# Autodesk Inventor assembly: Gearbox Assembly
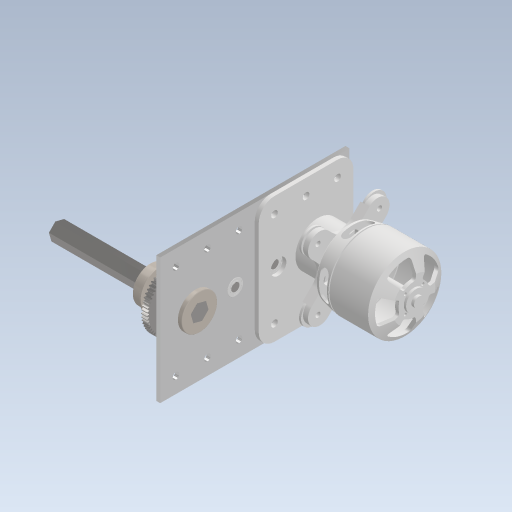
[picture p0: Inventor's stored thumbnail of the model, 512x512]
Saved by Autodesk Inventor 2023 (Build 270158000, 158)
## iProperties
Created: 2023-02-14
Part Number: Gearbox Assembly
Document SubType Name: Assembly
Designer: Dave
Mass: 682.162 g
Surface Area: 1267.39 cm^2
Volume: 183.282 cm^3
Density: 3.72192 g/cm^3
Author: Dave
## Documents named in this file (14)
- C:\Users\Dave\Documents\GitHub\BehrendURCMechanical\CAD\Chassis\GearBox\Final Gears and Assemblies\Gearbox Assembly.iam
- C:\Users\Dave\Documents\GitHub\BehrendURCMechanical\CAD\Chassis\GearBox\Final Gears and Assemblies\CH-1-01-20T_Drive Gear.ipt
- C:\Users\Dave\Documents\GitHub\BehrendURCMechanical\CAD\Chassis\GearBox\Final Gears and Assemblies\CH-1-01-60T_Output.ipt
- C:\Users\Dave\Documents\GitHub\BehrendURCMechanical\CAD\Chassis\GearBox\Final Gears and Assemblies\CH-1-01-20T_Idler.ipt
- C:\Users\Dave\Documents\GitHub\BehrendURCMechanical\CAD\Chassis\GearBox\Final Gears and Assemblies\CH-1-01-60T_Idler.ipt
- C:\Users\Dave\Documents\GitHub\BehrendURCMechanical\CAD\Chassis\GearBox\Housing\CH-1-02-RearGearboxHousingMotorSide.ipt
- C:\Users\Dave\Documents\GitHub\BehrendURCMechanical\CAD\Chassis\GearBox\Drive Motor Shaft Coupler.ipt
- C:\Users\Dave\Documents\GitHub\BehrendURCMechanical\CAD\Chassis\GearBox\Drive Motor.ipt
- C:\Users\Dave\Documents\GitHub\BehrendURCMechanical\CAD\Chassis\GearBox\Ch-1-01-0.5x4.5HexShaft.ipt
- C:\Users\Dave\Documents\GitHub\BehrendURCMechanical\CAD\Chassis\GearBox\CH-1-01-0.25x1.875SmoothShaft.ipt
- C:\Users\Dave\Documents\GitHub\BehrendURCMechanical\CAD\Chassis\GearBox\CH-1-01-0.5HexBearing.ipt
- C:\Users\Dave\Documents\GitHub\BehrendURCMechanical\CAD\Chassis\GearBox\CH-1-01-0.25IDSmoothBoreBearing.ipt
- C:\Users\Dave\Documents\GitHub\BehrendURCMechanical\CAD\Chassis V3\DriveMotorPlate.ipt
- C:\Users\Dave\Documents\GitHub\BehrendURCMechanical\CAD\Chassis V3\DriveMotorMount2.ipt
## Components (21 placed, 13 different names)
1. CH-1-01-20T_Drive Gear:1 — Insert:3
2. CH-1-01-60T_Output:1 — Mate:17, Flush:6
3. CH-1-01-20T_Idler:1 — Mate:21, Flush:5
4. CH-1-01-60T_Idler:1 — Mate:18, Mate:19, Mate:20, Flush:5
5. CH-1-01-20T_Idler:2 — Mate:19, Mate:22, Flush:6
6. CH-1-01-60T_Idler:2 — Mate:10, Mate:11, Mate:23
7. CH-1-02-RearGearboxHousingMotorSide:1 — Angle:1, Flush:1, Flush:2, Insert:6, Insert:7, Insert:10, Mate:26, Angle:2, Flush:8, Flush:9
8. CH-1-02-RearGearboxHousingMotorSide:2 — Flush:1, Flush:2, Insert:8, Insert:9, Insert:11
9. Drive Motor Shaft Coupler:1 — Insert:3, Mate:23, Mate:24, Mate:25, Flush:7, Mate:26
10. Drive Motor:1 — Mate:24, Mate:25, Angle:2, Insert:14, Insert:15
11. Ch-1-01-0.5x4.5HexShaft:1 — Flush:3, Mate:8, Mate:9
12. CH-1-01-0.25x1.875SmoothShaft:1 — Insert:13
13. CH-1-01-0.25x1.875SmoothShaft:2 — Insert:12, Flush:4
14. CH-1-01-0.5HexBearing:1 — Insert:11, Mate:17
15. CH-1-01-0.5HexBearing:2 — Insert:10, Flush:3, Mate:8, Mate:9
16. CH-1-01-0.25IDSmoothBoreBearing:1 — Insert:6, Insert:12, Flush:7
17. CH-1-01-0.25IDSmoothBoreBearing:2 — Insert:7, Insert:13, Mate:11
18. CH-1-01-0.25IDSmoothBoreBearing:3 — Insert:8, Flush:4, Mate:18, Mate:20, Mate:22
19. CH-1-01-0.25IDSmoothBoreBearing:4 — Insert:9, Mate:10, Mate:21
20. DriveMotorPlate:1 — Insert:14, Insert:15, Flush:10
21. DriveMotorMount2:1 — Flush:8, Flush:9, Flush:10
## Relationships (37: Mate 14, Insert 11, Flush 10, Angle 2)
- Insert:3: CH-1-01-20T_Drive Gear:1 ↔ Drive Motor Shaft Coupler:1
- Angle:1 (0 deg): CH-1-02-RearGearboxHousingMotorSide:1
- Flush:1: CH-1-02-RearGearboxHousingMotorSide:1 ↔ CH-1-02-RearGearboxHousingMotorSide:2
- Flush:2: CH-1-02-RearGearboxHousingMotorSide:1 ↔ CH-1-02-RearGearboxHousingMotorSide:2
- Insert:6: CH-1-02-RearGearboxHousingMotorSide:1 ↔ CH-1-01-0.25IDSmoothBoreBearing:1
- Insert:7: CH-1-02-RearGearboxHousingMotorSide:1 ↔ CH-1-01-0.25IDSmoothBoreBearing:2
- Insert:8: CH-1-02-RearGearboxHousingMotorSide:2 ↔ CH-1-01-0.25IDSmoothBoreBearing:3
- Insert:9: CH-1-02-RearGearboxHousingMotorSide:2 ↔ CH-1-01-0.25IDSmoothBoreBearing:4
- Insert:10: CH-1-02-RearGearboxHousingMotorSide:1 ↔ CH-1-01-0.5HexBearing:2
- Insert:11: CH-1-02-RearGearboxHousingMotorSide:2 ↔ CH-1-01-0.5HexBearing:1
- Flush:3: Ch-1-01-0.5x4.5HexShaft:1 ↔ CH-1-01-0.5HexBearing:2
- Mate:8: Ch-1-01-0.5x4.5HexShaft:1 ↔ CH-1-01-0.5HexBearing:2
- Mate:9: Ch-1-01-0.5x4.5HexShaft:1 ↔ CH-1-01-0.5HexBearing:2
- Insert:12: CH-1-01-0.25x1.875SmoothShaft:2 ↔ CH-1-01-0.25IDSmoothBoreBearing:1
- Insert:13: CH-1-01-0.25x1.875SmoothShaft:1 ↔ CH-1-01-0.25IDSmoothBoreBearing:2
- Mate:10: CH-1-01-60T_Idler:2 ↔ CH-1-01-0.25IDSmoothBoreBearing:4
- Mate:11: CH-1-01-60T_Idler:2 ↔ CH-1-01-0.25IDSmoothBoreBearing:2
- Flush:4: CH-1-01-0.25x1.875SmoothShaft:2 ↔ CH-1-01-0.25IDSmoothBoreBearing:3
- Mate:17: CH-1-01-60T_Output:1 ↔ CH-1-01-0.5HexBearing:1
- Mate:18: CH-1-01-60T_Idler:1 ↔ CH-1-01-0.25IDSmoothBoreBearing:3
- Mate:19: CH-1-01-60T_Idler:1 ↔ CH-1-01-20T_Idler:2
- Mate:20: CH-1-01-60T_Idler:1 ↔ CH-1-01-0.25IDSmoothBoreBearing:3
- Mate:21: CH-1-01-20T_Idler:1 ↔ CH-1-01-0.25IDSmoothBoreBearing:4
- Flush:5: CH-1-01-20T_Idler:1 ↔ CH-1-01-60T_Idler:1
- Mate:22: CH-1-01-20T_Idler:2 ↔ CH-1-01-0.25IDSmoothBoreBearing:3
- Flush:6: CH-1-01-60T_Output:1 ↔ CH-1-01-20T_Idler:2
- Mate:23: CH-1-01-60T_Idler:2 ↔ Drive Motor Shaft Coupler:1
- Mate:24: Drive Motor Shaft Coupler:1 ↔ Drive Motor:1
- Mate:25: Drive Motor Shaft Coupler:1 ↔ Drive Motor:1
- Flush:7: Drive Motor Shaft Coupler:1 ↔ CH-1-01-0.25IDSmoothBoreBearing:1
- Mate:26: CH-1-02-RearGearboxHousingMotorSide:1 ↔ Drive Motor Shaft Coupler:1
- Angle:2 (0 deg): CH-1-02-RearGearboxHousingMotorSide:1 ↔ Drive Motor:1
- Insert:14: Drive Motor:1 ↔ DriveMotorPlate:1
- Insert:15: Drive Motor:1 ↔ DriveMotorPlate:1
- Flush:8: CH-1-02-RearGearboxHousingMotorSide:1 ↔ DriveMotorMount2:1
- Flush:9: CH-1-02-RearGearboxHousingMotorSide:1 ↔ DriveMotorMount2:1
- Flush:10: DriveMotorPlate:1 ↔ DriveMotorMount2:1
